# Autodesk Inventor assembly: ARM_ASSEMBLY
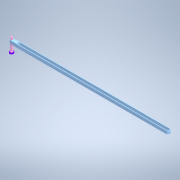
[picture p0: Inventor's stored thumbnail of the model, 180x180]
Saved by Autodesk Inventor 2022 (Build 260153000, 153)
## iProperties
Created: 2022-11-14
Part Number: ARM_ASSEMBLY
Document SubType Name: Assembly
Designer: matia
Author: matia
## Documents named in this file (4)
- C:\Users\matia\Desktop\1QuadMod\ARM_ASSEMBLY.iam
- C:\Users\matia\Desktop\1QuadMod\arm connector.ipt
- C:\Users\matia\Desktop\1QuadMod\ARMCONNECTORPLASTICBUSHING.ipt
- C:\Users\matia\Desktop\1QuadMod\arm.ipt
## Components (3 placed, 3 different names)
1. arm connector:1 — Mate:1, Mate:2, Mate:3
2. ARMCONNECTORPLASTICBUSHING:1 — Mate:1, Mate:2
3. arm:1 — Mate:3
## Relationships (3: Mate 3)
- Mate:1: arm connector:1 ↔ ARMCONNECTORPLASTICBUSHING:1
- Mate:2: arm connector:1 ↔ ARMCONNECTORPLASTICBUSHING:1
- Mate:3: arm connector:1 ↔ arm:1
